# Autodesk Inventor assembly: MBD_Rmotorbar
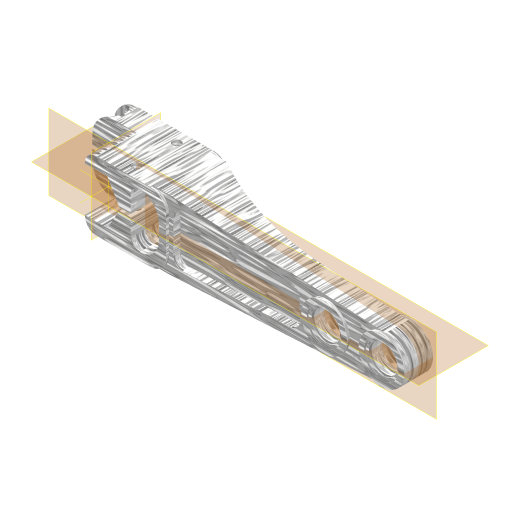
[picture p0: Inventor's stored thumbnail of the model, 512x512]
Saved by Autodesk Inventor 2023 (Build 270158000, 158)
## iProperties
Created: 2022-06-22
Part Number: MBD_Rmotorbar
Document SubType Name: Assembly
Designer: BioRoLaT470S
Mass: 51.906 g
Surface Area: 121.197 cm^2
Volume: 18.4719 cm^3
Density: 2.81 g/cm^3
Author: BioRoLaT470S
## Documents named in this file (2)
- C:\Users\guanlunlu\Desktop\MBD_CORGI\CAD\MBD_Rmotorbar.iam
- C:\Users\guanlunlu\Desktop\MBD_CORGI\R100_properties\組合檔_v4\Lmotor_v3(open).ipt
## Components (1 placed, 1 different names)
1. Lmotor_v3(open):1 — Mate:1, Flush:1, Flush:2
## Relationships (3: Flush 2, Mate 1)
- Mate:1: Lmotor_v3(open):1
- Flush:1: Lmotor_v3(open):1
- Flush:2: Lmotor_v3(open):1
